# Autodesk Inventor assembly: finger 4
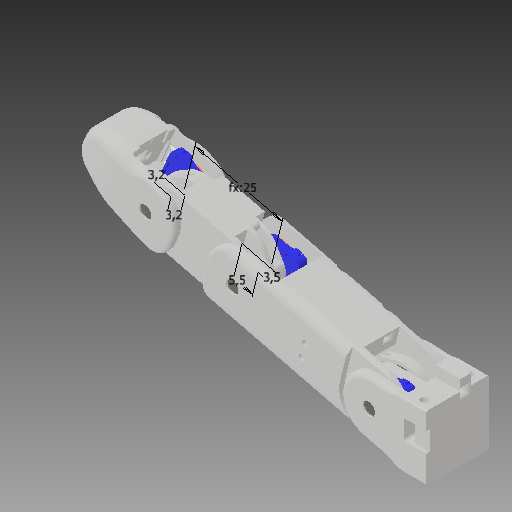
[picture p0: Inventor's stored thumbnail of the model, 512x512]
Saved by Autodesk Inventor 2017 SP1 (Build 210196100, 196)
## iProperties
Created: 2018-09-01
Part Number: finger 4
Document SubType Name: Assembly
Designer: jakub.tomczynski
Author: jakub.tomczynski
## Documents named in this file (22)
- C:\InventorVault-Lider\LiderWorkspace\LiderHand\underactuated finger\finger 4.iam
- C:\InventorVault-Lider\LiderWorkspace\LiderHand\underactuated finger\MCP mount L.ipt
- C:\InventorVault-Lider\LiderWorkspace\LiderHand\underactuated finger\MCP mount M F4.ipt
- C:\InventorVault-Lider\LiderWorkspace\LiderHand\underactuated finger\MCP mount R.ipt
- C:\InventorVault-Lider\LiderWorkspace\LiderHand\underactuated finger\MCP axle.ipt
- C:\InventorVault-Lider\LiderWorkspace\LiderHand\underactuated finger\phalanx 1 L F4.ipt
- C:\InventorVault-Lider\LiderWorkspace\LiderHand\underactuated finger\phalanx 1 R F4.ipt
- C:\InventorVault-Lider\LiderWorkspace\LiderHand\underactuated finger\IP axle.ipt
- C:\InventorVault-Lider\LiderWorkspace\LiderHand\underactuated finger\phalanx 2 L F4.ipt
- C:\InventorVault-Lider\LiderWorkspace\LiderHand\underactuated finger\phalanx 2 R F4.ipt
- C:\InventorVault-Lider\LiderWorkspace\LiderHand\underactuated finger\phalanx 3 L.ipt
- C:\InventorVault-Lider\LiderWorkspace\LiderHand\underactuated finger\tendon anchor.ipt
- C:\InventorVault-Lider\LiderWorkspace\LiderHand\underactuated finger\phalanx 3 R.ipt
- C:\InventorVault-Lider\LiderWorkspace\LiderHand\underactuated finger\phalanx 3 spring pins support.ipt
- C:\InventorVault-Lider\LiderWorkspace\LiderHand\parts\bearing_2x5x1,5.ipt
- C:\InventorVault-Lider\LiderWorkspace\LiderHand\parts\alps_RDC503013A.ipt
- C:\InventorVault-Lider\LiderWorkspace\LiderHand\parts\bearing_6x10x2,5.ipt
- C:\InventorVault-Lider\LiderWorkspace\LiderHand\parts\bearing_7x11x2,5.ipt
- C:\InventorVault-Lider\LiderWorkspace\LiderHand\underactuated finger\double spring swivel 6.ipt
- C:\InventorVault-Lider\LiderWorkspace\LiderHand\underactuated finger\double spring swivel 7.ipt
- C:\InventorVault-Lider\LiderWorkspace\LiderHand\parts\pin 1.5x7.8.ipt
- C:\InventorVault-Lider\LiderWorkspace\LiderHand\parts\pin 1.5x5.8.ipt
## Components (33 placed, 21 different names)
1. MCP mount L:1 — Flush:1, Flush:2, Flush:3, Mate:1, Mate:2, Mate:3, Mate:5, Mate:6, Mate:8, Mate:9
2. MCP mount M F4:1 — Mate:1, Mate:2, Mate:3, Mate:4, Mate:64, Mate:65, Mate:66, Mate:67, Mate:68, Mate:83, Mate:86
3. MCP mount R:1 — Mate:4, Mate:5, Mate:6, Mate:7, Mate:10
4. bearing_2x5x1,5:7 — Mate:8, Mate:9, Mate:11, Mate:13
5. bearing_2x5x1,5:8 — Mate:7, Mate:10, Mate:12, Mate:14
6. MCP axle:1 — Mate:11, Mate:12, Mate:13, Mate:14, Mate:20, Mate:21, Mate:22, Mate:23, Mate:24, Mate:63
7. phalanx 1 L F4:1 — Mate:15, Mate:16, Mate:17, Mate:18, Mate:19, Mate:22, Mate:23, Mate:26, Mate:28, Mate:71, Mate:72, Mate:73, Mate:74, Mate:75, Angle:1, Angle:2, Mate:90, Mate:91, Mate:92, Mate:93
8. phalanx 1 R F4:1 — Mate:15, Mate:16, Mate:17, Mate:18, Mate:19, Mate:20, Mate:21, Mate:24, Mate:25, Mate:27
9. bearing_2x5x1,5:9 — Mate:25, Mate:27, Mate:30, Mate:31
10. bearing_2x5x1,5:10 — Mate:26, Mate:28, Mate:29, Mate:32
11. IP axle:1 — Mate:29, Mate:30, Mate:31, Mate:32, Mate:36, Mate:37, Mate:38, Mate:39, Mate:40, Mate:69
12. phalanx 2 L F4:1 — Mate:33, Mate:34, Mate:35, Mate:37, Mate:38, Mate:40, Mate:41, Mate:43, Mate:45
13. phalanx 2 R F4:1 — Mate:33, Mate:34, Mate:35, Mate:36, Mate:39, Mate:42, Mate:44, Mate:81, Mate:82, Mate:84, Mate:85
14. IP axle:2 — Mate:41, Mate:42, Mate:43, Mate:44, Mate:45, Mate:48, Mate:49, Mate:55, Mate:56, Mate:70
15. phalanx 3 L:1 — Mate:46, Mate:47, Mate:50, Mate:51, Mate:52, Mate:53, Mate:54, Mate:58, Mate:76, Mate:77, Mate:78, Mate:79, Mate:80, Angle:3
16. bearing_2x5x1,5:11 — Mate:46, Mate:47, Mate:48, Mate:49
17. tendon anchor:1 — Mate:50, Mate:51, Mate:52
18. phalanx 3 R:1 — Mate:53, Mate:54, Mate:57, Mate:58, Mate:59, Mate:60, Mate:61, Mate:62, Mate:94, Mate:95, Mate:96, Mate:97
19. bearing_2x5x1,5:12 — Mate:55, Mate:56, Mate:57, Mate:59
20. phalanx 3 spring pins support:1 — Mate:60, Mate:61, Mate:62
21. alps_RDC503013A:1 — Mate:70, Mate:76, Mate:77, Mate:78, Mate:79, Mate:80
22. alps_RDC503013A:2 — Mate:69, Mate:71, Mate:72, Mate:73, Mate:74, Mate:75
23. alps_RDC503013A:3 — Mate:63, Mate:64, Mate:65, Mate:66, Mate:67, Mate:68
24. bearing_6x10x2,5:1 — Mate:81, Mate:84, Mate:88, Flush:4
25. bearing_7x11x2,5:1 — Mate:83, Mate:86, Mate:89, Flush:6
26. bearing_6x10x2,5:2 — Mate:82, Mate:85, Mate:87, Flush:5
27. double spring swivel 6:1 — Mate:87, Flush:5, Angle:2
28. double spring swivel 7:1 — Mate:89, Flush:6, Angle:1
29. double spring swivel 6:2 — Mate:88, Flush:4, Angle:3
30. pin 1.5x7.8:1 — Mate:90, Mate:92
31. pin 1.5x7.8:2 — Mate:91, Mate:93
32. pin 1.5x5.8:1 — Mate:94, Mate:96
33. pin 1.5x5.8:2 — Mate:95, Mate:97
## Relationships (106: Mate 97, Flush 6, Angle 3)
- Flush:1: MCP mount L:1
- Flush:2: MCP mount L:1
- Flush:3: MCP mount L:1
- Mate:1: MCP mount L:1 ↔ MCP mount M F4:1
- Mate:2: MCP mount L:1 ↔ MCP mount M F4:1
- Mate:3: MCP mount L:1 ↔ MCP mount M F4:1
- Mate:4: MCP mount M F4:1 ↔ MCP mount R:1
- Mate:5: MCP mount L:1 ↔ MCP mount R:1
- Mate:6: MCP mount L:1 ↔ MCP mount R:1
- Mate:7: MCP mount R:1 ↔ bearing_2x5x1,5:8
- Mate:8: MCP mount L:1 ↔ bearing_2x5x1,5:7
- Mate:9: MCP mount L:1 ↔ bearing_2x5x1,5:7
- Mate:10: MCP mount R:1 ↔ bearing_2x5x1,5:8
- Mate:11: bearing_2x5x1,5:7 ↔ MCP axle:1
- Mate:12: bearing_2x5x1,5:8 ↔ MCP axle:1
- Mate:13: bearing_2x5x1,5:7 ↔ MCP axle:1
- Mate:14: bearing_2x5x1,5:8 ↔ MCP axle:1
- Mate:15: phalanx 1 L F4:1 ↔ phalanx 1 R F4:1
- Mate:16: phalanx 1 L F4:1 ↔ phalanx 1 R F4:1
- Mate:17: phalanx 1 L F4:1 ↔ phalanx 1 R F4:1
- Mate:18: phalanx 1 L F4:1 ↔ phalanx 1 R F4:1
- Mate:19: phalanx 1 L F4:1 ↔ phalanx 1 R F4:1
- Mate:20: MCP axle:1 ↔ phalanx 1 R F4:1
- Mate:21: MCP axle:1 ↔ phalanx 1 R F4:1
- Mate:22: MCP axle:1 ↔ phalanx 1 L F4:1
- Mate:23: MCP axle:1 ↔ phalanx 1 L F4:1
- Mate:24: MCP axle:1 ↔ phalanx 1 R F4:1
- Mate:25: phalanx 1 R F4:1 ↔ bearing_2x5x1,5:9
- Mate:26: phalanx 1 L F4:1 ↔ bearing_2x5x1,5:10
- Mate:27: phalanx 1 R F4:1 ↔ bearing_2x5x1,5:9
- Mate:28: phalanx 1 L F4:1 ↔ bearing_2x5x1,5:10
- Mate:29: bearing_2x5x1,5:10 ↔ IP axle:1
- Mate:30: bearing_2x5x1,5:9 ↔ IP axle:1
- Mate:31: bearing_2x5x1,5:9 ↔ IP axle:1
- Mate:32: bearing_2x5x1,5:10 ↔ IP axle:1
- Mate:33: phalanx 2 L F4:1 ↔ phalanx 2 R F4:1
- Mate:34: phalanx 2 L F4:1 ↔ phalanx 2 R F4:1
- Mate:35: phalanx 2 L F4:1 ↔ phalanx 2 R F4:1
- Mate:36: IP axle:1 ↔ phalanx 2 R F4:1
- Mate:37: IP axle:1 ↔ phalanx 2 L F4:1
- Mate:38: IP axle:1 ↔ phalanx 2 L F4:1
- Mate:39: IP axle:1 ↔ phalanx 2 R F4:1
- Mate:40: IP axle:1 ↔ phalanx 2 L F4:1
- Mate:41: phalanx 2 L F4:1 ↔ IP axle:2
- Mate:42: phalanx 2 R F4:1 ↔ IP axle:2
- Mate:43: phalanx 2 L F4:1 ↔ IP axle:2
- Mate:44: phalanx 2 R F4:1 ↔ IP axle:2
- Mate:45: phalanx 2 L F4:1 ↔ IP axle:2
- Mate:46: phalanx 3 L:1 ↔ bearing_2x5x1,5:11
- Mate:47: phalanx 3 L:1 ↔ bearing_2x5x1,5:11
- Mate:48: IP axle:2 ↔ bearing_2x5x1,5:11
- Mate:49: IP axle:2 ↔ bearing_2x5x1,5:11
- Mate:50: phalanx 3 L:1 ↔ tendon anchor:1
- Mate:51: phalanx 3 L:1 ↔ tendon anchor:1
- Mate:52: phalanx 3 L:1 ↔ tendon anchor:1
- Mate:53: phalanx 3 L:1 ↔ phalanx 3 R:1
- Mate:54: phalanx 3 L:1 ↔ phalanx 3 R:1
- Mate:55: IP axle:2 ↔ bearing_2x5x1,5:12
- Mate:56: IP axle:2 ↔ bearing_2x5x1,5:12
- Mate:57: phalanx 3 R:1 ↔ bearing_2x5x1,5:12
- Mate:58: phalanx 3 L:1 ↔ phalanx 3 R:1
- Mate:59: phalanx 3 R:1 ↔ bearing_2x5x1,5:12
- Mate:60: phalanx 3 R:1 ↔ phalanx 3 spring pins support:1
- Mate:61: phalanx 3 R:1 ↔ phalanx 3 spring pins support:1
- Mate:62: phalanx 3 R:1 ↔ phalanx 3 spring pins support:1
- Mate:63: MCP axle:1 ↔ alps_RDC503013A:3
- Mate:64: MCP mount M F4:1 ↔ alps_RDC503013A:3
- Mate:65: MCP mount M F4:1 ↔ alps_RDC503013A:3
- Mate:66: MCP mount M F4:1 ↔ alps_RDC503013A:3
- Mate:67: MCP mount M F4:1 ↔ alps_RDC503013A:3
- Mate:68: MCP mount M F4:1 ↔ alps_RDC503013A:3
- Mate:69: IP axle:1 ↔ alps_RDC503013A:2
- Mate:70: IP axle:2 ↔ alps_RDC503013A:1
- Mate:71: phalanx 1 L F4:1 ↔ alps_RDC503013A:2
- Mate:72: phalanx 1 L F4:1 ↔ alps_RDC503013A:2
- Mate:73: phalanx 1 L F4:1 ↔ alps_RDC503013A:2
- Mate:74: phalanx 1 L F4:1 ↔ alps_RDC503013A:2
- Mate:75: phalanx 1 L F4:1 ↔ alps_RDC503013A:2
- Mate:76: phalanx 3 L:1 ↔ alps_RDC503013A:1
- Mate:77: phalanx 3 L:1 ↔ alps_RDC503013A:1
- Mate:78: phalanx 3 L:1 ↔ alps_RDC503013A:1
- Mate:79: phalanx 3 L:1 ↔ alps_RDC503013A:1
- Mate:80: phalanx 3 L:1 ↔ alps_RDC503013A:1
- Mate:81: phalanx 2 R F4:1 ↔ bearing_6x10x2,5:1
- Mate:82: phalanx 2 R F4:1 ↔ bearing_6x10x2,5:2
- Mate:83: MCP mount M F4:1 ↔ bearing_7x11x2,5:1
- Mate:84: phalanx 2 R F4:1 ↔ bearing_6x10x2,5:1
- Mate:85: phalanx 2 R F4:1 ↔ bearing_6x10x2,5:2
- Mate:86: MCP mount M F4:1 ↔ bearing_7x11x2,5:1
- Mate:87: bearing_6x10x2,5:2 ↔ double spring swivel 6:1
- Mate:88: bearing_6x10x2,5:1 ↔ double spring swivel 6:2
- Mate:89: bearing_7x11x2,5:1 ↔ double spring swivel 7:1
- Flush:4: bearing_6x10x2,5:1 ↔ double spring swivel 6:2
- Flush:5: bearing_6x10x2,5:2 ↔ double spring swivel 6:1
- Flush:6: bearing_7x11x2,5:1 ↔ double spring swivel 7:1
- Angle:1 (180 deg): phalanx 1 L F4:1 ↔ double spring swivel 7:1
- Angle:2 (0 deg): phalanx 1 L F4:1 ↔ double spring swivel 6:1
- Angle:3 (180 deg): phalanx 3 L:1 ↔ double spring swivel 6:2
- Mate:90: phalanx 1 L F4:1 ↔ pin 1.5x7.8:1
- Mate:91: phalanx 1 L F4:1 ↔ pin 1.5x7.8:2
- Mate:92: phalanx 1 L F4:1 ↔ pin 1.5x7.8:1
- Mate:93: phalanx 1 L F4:1 ↔ pin 1.5x7.8:2
- Mate:94: phalanx 3 R:1 ↔ pin 1.5x5.8:1
- Mate:95: phalanx 3 R:1 ↔ pin 1.5x5.8:2
- Mate:96: phalanx 3 R:1 ↔ pin 1.5x5.8:1
- Mate:97: phalanx 3 R:1 ↔ pin 1.5x5.8:2
